# Autodesk Inventor assembly: MAN_ASSEMBLY
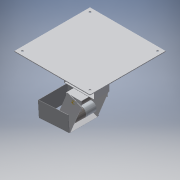
[picture p0: Inventor's stored thumbnail of the model, 180x180]
Saved by Autodesk Inventor 2019 (Build 230136000, 136)
## iProperties
Created: 2021-03-06
Part Number: MAN_ASSEMBLY
Document SubType Name: Assembly
Designer: DOMEK
Author: DOMEK
## Documents named in this file (7)
- D:\Manipulator\Inventor\MAN_ASSEMBLY.iam
- D:\Manipulator\Inventor\MAN_BASIS_PLATE.ipt
- D:\Manipulator\Inventor\MAN_BASIS_PRIMARY_STRUCTURE.ipt
- D:\Manipulator\Inventor\MAN_BASIS_SECONDARY_STRUCTURE.ipt
- D:\Manipulator\Inventor\25d-gearmotor-3d-models\25d-metal-gearmotor-378-499-encoder.ipt
- D:\Manipulator\Inventor\MAN_SERVO_HANDLER.ipt
- D:\Manipulator\Inventor\MAN_BASIS_THIRD_STRUCTURE.ipt
## Components (8 placed, 6 different names)
1. MAN_BASIS_PLATE:1 — Mate:1
2. MAN_BASIS_PRIMARY_STRUCTURE:1 — Mate:1, Mate:2, Insert:3
3. 25d-metal-gearmotor-378-499-encoder:1 — Mate:2, Insert:3, Insert:4
4. MAN_SERVO_HANDLER:1 — Insert:4, Insert:5
5. 25d-metal-gearmotor-378-499-encoder:2 — Insert:5, Insert:6
6. MAN_BASIS_THIRD_STRUCTURE:1 — Insert:6, Insert:7
7. 25d-metal-gearmotor-378-499-encoder:3 — Insert:7, Insert:8
8. MAN_BASIS_SECONDARY_STRUCTURE:1 — Insert:8
## Relationships (8: Insert 6, Mate 2)
- Mate:1: MAN_BASIS_PLATE:1 ↔ MAN_BASIS_PRIMARY_STRUCTURE:1
- Mate:2 (8 mm): MAN_BASIS_PRIMARY_STRUCTURE:1 ↔ 25d-metal-gearmotor-378-499-encoder:1
- Insert:3: MAN_BASIS_PRIMARY_STRUCTURE:1 ↔ 25d-metal-gearmotor-378-499-encoder:1
- Insert:4 (-6 mm): 25d-metal-gearmotor-378-499-encoder:1 ↔ MAN_SERVO_HANDLER:1
- Insert:5 (-2 mm): MAN_SERVO_HANDLER:1 ↔ 25d-metal-gearmotor-378-499-encoder:2
- Insert:6 (-10 mm): 25d-metal-gearmotor-378-499-encoder:2 ↔ MAN_BASIS_THIRD_STRUCTURE:1
- Insert:7 (-12 mm): MAN_BASIS_THIRD_STRUCTURE:1 ↔ 25d-metal-gearmotor-378-499-encoder:3
- Insert:8 (-8 mm): 25d-metal-gearmotor-378-499-encoder:3 ↔ MAN_BASIS_SECONDARY_STRUCTURE:1
